# Autodesk Inventor assembly: Rotor assembly for 250W servo
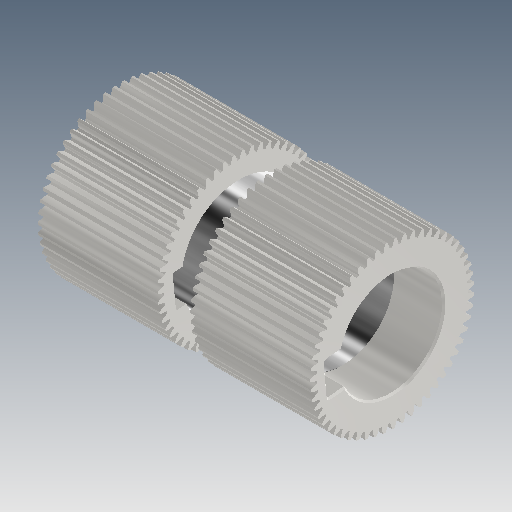
[picture p0: Inventor's stored thumbnail of the model, 512x512]
Saved by Autodesk Inventor 2020.3 (Build 243373010, 373A)
## iProperties
Created: 2021-04-26
Part Number: Rotor assembly for 250W servo
Document SubType Name: Assembly
Designer: marti
Author: marti
## Documents named in this file (3)
- C:\Users\marti\Documents\Inventor\RobotManipulateArm\17.4.2021 - Complete new IDEA\Servo\Rotor assembly for 250W servo.iam
- C:\Users\marti\Documents\Inventor\RobotManipulateArm\17.4.2021 - Complete new IDEA\Servo\Rotor for 250W servo.iam
- C:\Users\marti\Documents\Inventor\RobotManipulateArm\17.4.2021 - Complete new IDEA\Servo\Pernament magnet.ipt
## Components (3 placed, 2 different names)
1. Rotor for 250W servo:1 [sub-assembly] — Mate:1, Mate:6, Tangent:1, Mate:10
2. Rotor for 250W servo:3 [sub-assembly] — Mate:6, Tangent:1, Mate:7, Mate:8, Mate:9
3. Pernament magnet:2 — Mate:7, Mate:8, Mate:9, Mate:10
## Relationships (7: Mate 6, Tangent 1)
- Mate:1: Rotor for 250W servo:1
- Mate:6: Rotor for 250W servo:1 ↔ Rotor for 250W servo:3
- Tangent:1: Rotor for 250W servo:1 ↔ Rotor for 250W servo:3
- Mate:7: Rotor for 250W servo:3 ↔ Pernament magnet:2
- Mate:8: Rotor for 250W servo:3 ↔ Pernament magnet:2
- Mate:9: Rotor for 250W servo:3 ↔ Pernament magnet:2
- Mate:10: Rotor for 250W servo:1 ↔ Pernament magnet:2
